# Autodesk Inventor assembly: ExtendingArm_ProperConstraints
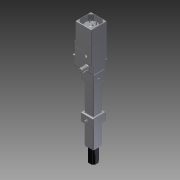
[picture p0: Inventor's stored thumbnail of the model, 180x180]
Saved by Autodesk Inventor 2012 (Build 160160000, 160)
## iProperties
Created: 2011-10-02
Part Number: ExtendingArm_ProperConstraints
Document SubType Name: Assembly
Designer: KuttaA
Mass: 266.79 g
Surface Area: 1474.69 cm^2
Volume: 266.518 cm^3
Density: 1.00102 g/cm^3
Author: KuttaA
## Documents named in this file (15)
- C:\Users\Drew\Dropbox\Hexapod Research\Leg Design\ExtendingArm_ProperConstraints.iam
- C:\Users\Drew\Dropbox\Hexapod Research\Leg Design\Screw.ipt
- C:\Users\Drew\Dropbox\Hexapod Research\Leg Design\LowerArm.ipt
- C:\Users\Drew\Dropbox\Hexapod Research\Leg Design\UpperRobotArm.ipt
- C:\Users\Drew\Dropbox\Hexapod Research\Leg Design\InternalKey.ipt
- C:\Users\Drew\Dropbox\Hexapod Research\Leg Design\Other Parts\Intermediary Gear Box\GearBox_ProperConstraints.iam
- C:\Users\Drew\Dropbox\Hexapod Research\Leg Design\Other Parts\Motor Housing\MotorHousingTopMotorSupport.ipt
- C:\Users\Drew\Dropbox\Hexapod Research\Leg Design\Other Parts\Motor Housing\MotorHousingGearboxTop.ipt
- C:\Users\Drew\Dropbox\Hexapod Research\Leg Design\Other Parts\MotorHousing.ipt
- C:\Users\Drew\Dropbox\Hexapod Research\Leg Design\Other Parts\ArmPivot.ipt
- C:\Users\Drew\Dropbox\Hexapod Research\Leg Design\Other Parts\Motor.ipt
- C:\Users\Drew\Dropbox\Hexapod Research\Leg Design\Other Parts\MotorToHexKey.ipt
- C:\Users\Drew\Dropbox\Hexapod Research\Leg Design\Other Parts\Motor Housing\MotorHousingBottom_split1.ipt
- C:\Users\Drew\Dropbox\Hexapod Research\Leg Design\Other Parts\Motor Housing\MotorHousingBottom_split2.ipt
- C:\Users\Drew\Dropbox\Hexapod Research\Leg Design\Other Parts\Motor Housing\MotorHousingBottom_split3.ipt
## Components (15 placed, 14 different names)
1. Screw:1 — Mate:1, Angle:1, Mate:2, Mate:3, Mate:10, Mate:11, Mate:24
2. LowerArm:1 — Mate:1, Angle:1, Angle:2, Flush:1
3. UpperRobotArm:1 — Mate:2, Mate:3, Angle:2, Mate:4, Mate:5, Mate:6, Mate:18, Mate:19, Flush:1, Angle:3, Mate:28
4. InternalKey:1 — Mate:4, Mate:5, Mate:6, Mate:27
5. GearBox_ProperConstraints:1 [sub-assembly] — Mate:10, Mate:11, Angle:5, Mate:32, Mate:33
6. MotorHousingTopMotorSupport:1 — Mate:35, Flush:5
7. MotorHousingGearboxTop:1 — Mate:36, Mate:38, Angle:6
8. ServoPivot — Mate:18, Mate:19, Mate:20, Mate:21, Mate:22, Mate:23
9. ArmPivot:1 — Mate:22, Mate:23
10. ArmPivot:2 — Mate:20, Mate:21
11. Motor:1 — Mate:25, Mate:29, Mate:30, Mate:31
12. MotorToHexKey:1 — Mate:25, Mate:32, Mate:33
13. MotorHousingBottom_split1:1 — Mate:29, Mate:30, Mate:31, Angle:4, Flush:2, Mate:34, Flush:4, Mate:35, Flush:5, Flush:6
14. MotorHousingBottom_split2:1 — Mate:27, Angle:3, Mate:28, Angle:4, Flush:2, Angle:5, Mate:34, Mate:37, Mate:38, Angle:6
15. MotorHousingBottom_split3:1 — Flush:4, Flush:6
## Relationships (39: Mate 28, Angle 6, Flush 5)
- Mate:1: Screw:1 ↔ LowerArm:1
- Angle:1 (0 deg): Screw:1 ↔ LowerArm:1
- Mate:2: Screw:1 ↔ UpperRobotArm:1
- Mate:3 (0.3 mm): Screw:1 ↔ UpperRobotArm:1
- Angle:2 (0 deg): LowerArm:1 ↔ UpperRobotArm:1
- Mate:4 (0.3 mm): UpperRobotArm:1 ↔ InternalKey:1
- Mate:5 (0.3 mm): UpperRobotArm:1 ↔ InternalKey:1
- Mate:6 (0.3 mm): UpperRobotArm:1 ↔ InternalKey:1
- Mate:10: Screw:1 ↔ GearBox_ProperConstraints:1
- Mate:11 (0.3 mm): Screw:1 ↔ GearBox_ProperConstraints:1
- Mate:18 (0.3 mm): UpperRobotArm:1 ↔ ServoPivot
- Mate:19 (0.3 mm): UpperRobotArm:1 ↔ ServoPivot
- Mate:20: ServoPivot ↔ ArmPivot:2
- Mate:21 (0.3 mm): ServoPivot ↔ ArmPivot:2
- Mate:22: ServoPivot ↔ ArmPivot:1
- Mate:23: ServoPivot ↔ ArmPivot:1
- Flush:1 (40.478 mm): LowerArm:1 ↔ UpperRobotArm:1
- Mate:24: Screw:1
- Mate:25: Motor:1 ↔ MotorToHexKey:1
- Mate:27: InternalKey:1 ↔ MotorHousingBottom_split2:1
- Angle:3 (180 deg): UpperRobotArm:1 ↔ MotorHousingBottom_split2:1
- Mate:28 (0.3 mm): UpperRobotArm:1 ↔ MotorHousingBottom_split2:1
- Mate:29: Motor:1 ↔ MotorHousingBottom_split1:1
- Mate:30: Motor:1 ↔ MotorHousingBottom_split1:1
- Mate:31: Motor:1 ↔ MotorHousingBottom_split1:1
- Angle:4 (180 deg): MotorHousingBottom_split1:1 ↔ MotorHousingBottom_split2:1
- Flush:2: MotorHousingBottom_split1:1 ↔ MotorHousingBottom_split2:1
- Angle:5 (180 deg): GearBox_ProperConstraints:1 ↔ MotorHousingBottom_split2:1
- Mate:32: GearBox_ProperConstraints:1 ↔ MotorToHexKey:1
- Mate:33: GearBox_ProperConstraints:1 ↔ MotorToHexKey:1
- Mate:34 (25.75 mm): MotorHousingBottom_split1:1 ↔ MotorHousingBottom_split2:1
- Flush:4: MotorHousingBottom_split1:1 ↔ MotorHousingBottom_split3:1
- Mate:35: MotorHousingTopMotorSupport:1 ↔ MotorHousingBottom_split1:1
- Flush:5: MotorHousingTopMotorSupport:1 ↔ MotorHousingBottom_split1:1
- Flush:6: MotorHousingBottom_split1:1 ↔ MotorHousingBottom_split3:1
- Mate:36: MotorHousingGearboxTop:1
- Mate:37: MotorHousingBottom_split2:1
- Mate:38 (0.3 mm): MotorHousingGearboxTop:1 ↔ MotorHousingBottom_split2:1
- Angle:6 (0 deg): MotorHousingGearboxTop:1 ↔ MotorHousingBottom_split2:1
